# Autodesk Inventor assembly: NASA-20-FR
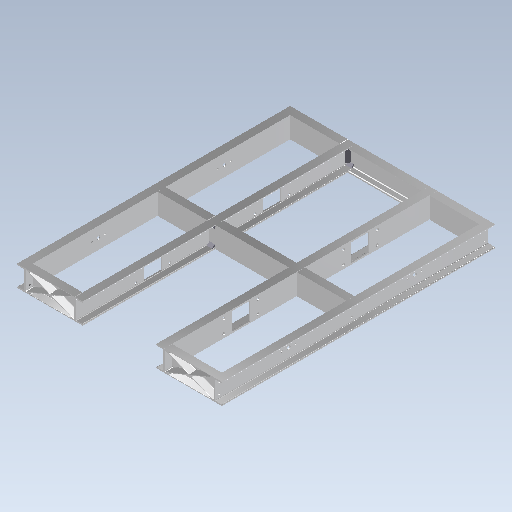
[picture p0: Inventor's stored thumbnail of the model, 512x512]
Saved by Autodesk Inventor 2020 (Build 240168000, 168)
## iProperties
Created: 2019-09-07
Part Number: NASA-20-FR
Document SubType Name: Weldment
Designer: Rick Szalay
Weld Material: Welded Aluminum-6061
Author: Rick Szalay
## Documents named in this file (6)
- C:\Users\Rick Szalay\Documents\NASA-20\NASA-20\FR\NASA-20-FR.iam
- C:\Users\Rick Szalay\Documents\NASA-20\NASA-20\FR\NASA-20-FR-SP-01.ipt
- C:\Users\Rick Szalay\Documents\NASA-20\NASA-20\FR\NASA-20-FR-BK-01.ipt
- C:\Users\Rick Szalay\Documents\NASA-20\NASA-20\FR\NASA-20-FR-FP-01.ipt
- C:\Users\Rick Szalay\Documents\NASA-20\NASA-20\FR\NASA-20-FR-TB-01.ipt
- C:\Users\Rick Szalay\Documents\NASA-20\NASA-20\FR\NASA-20-OP-01.ipt
## Components (12 placed, 5 different names)
1. NASA-20-FR-TB-01:1
2. NASA-20-FR-TB-01:2
3. NASA-20-FR-TB-01:3 — Flush:19
4. NASA-20-FR-TB-01:4
5. NASA-20-FR-TB-01:5 — Flush:18
6. NASA-20-FR-TB-01:6
7. NASA-20-FR-SP-01:1 — Mate:3, Mate:4
8. NASA-20-FR-SP-01:2 — Mate:3
9. NASA-20-FR-BK-01:1 — Flush:7, Mate:5
10. NASA-20-FR-FP-01:1 — Mate:5, Flush:18, Flush:19
11. NASA-20-OP-01:2
12. NASA-20-OP-01:1
## Relationships (35: Flush 22, Mate 13)
- [Flush]: NASA-20-FR-SP-01:1 ↔ NASA-20-FR-SP-01:2
- [Flush]: NASA-20-FR-SP-01:1 ↔ NASA-20-FR-SP-01:2
- [Flush]: NASA-20-FR-SP-01:1 ↔ NASA-20-FR-BK-01:1
- [Flush]: NASA-20-FR-SP-01:1 ↔ NASA-20-FR-BK-01:1
- [Mate]: NASA-20-FR-SP-01:1 ↔ NASA-20-FR-BK-01:1
- [Mate]: NASA-20-FR-SP-01:1 ↔ NASA-20-FR-FP-01:1
- [Flush]: NASA-20-FR-SP-01:1 ↔ NASA-20-FR-FP-01:1
- Mate:3 (-215.9 mm): NASA-20-FR-SP-01:1 ↔ NASA-20-FR-SP-01:2
- Mate:4: NASA-20-FR-SP-01:1
- Flush:7: NASA-20-FR-BK-01:1
- Mate:5 (-339.725 mm): NASA-20-FR-BK-01:1 ↔ NASA-20-FR-FP-01:1
- [Mate]: NASA-20-FR-TB-01:1 ↔ NASA-20-FR-SP-01:2
- [Flush]: NASA-20-FR-TB-01:1 ↔ NASA-20-FR-BK-01:1
- [Flush]: NASA-20-FR-TB-01:1 ↔ NASA-20-FR-SP-01:2
- [Mate]: NASA-20-FR-TB-01:3 ↔ NASA-20-FR-SP-01:2
- [Flush]: NASA-20-FR-TB-01:3 ↔ NASA-20-FR-SP-01:2
- [Mate]: NASA-20-FR-TB-01:2 ↔ NASA-20-FR-SP-01:2
- [Flush]: NASA-20-FR-TB-01:2 ↔ NASA-20-FR-SP-01:2
- [Flush]: NASA-20-FR-TB-01:2 ↔ NASA-20-FR-SP-01:2
- [Mate]: NASA-20-FR-TB-01:6 ↔ NASA-20-FR-SP-01:1
- [Mate]: NASA-20-FR-TB-01:5 ↔ NASA-20-FR-SP-01:1
- [Mate]: NASA-20-FR-TB-01:4 ↔ NASA-20-FR-SP-01:1
- [Flush]: NASA-20-FR-TB-01:5 ↔ NASA-20-FR-SP-01:1
- [Flush]: NASA-20-FR-TB-01:6 ↔ NASA-20-FR-BK-01:1
- [Flush]: NASA-20-FR-TB-01:4 ↔ NASA-20-FR-SP-01:1
- [Flush]: NASA-20-FR-TB-01:4 ↔ NASA-20-FR-SP-01:1
- [Flush]: NASA-20-FR-TB-01:6 ↔ NASA-20-FR-BK-01:1
- Flush:18: NASA-20-FR-TB-01:5 ↔ NASA-20-FR-FP-01:1
- Flush:19: NASA-20-FR-TB-01:3 ↔ NASA-20-FR-FP-01:1
- [Flush]: NASA-20-OP-01:2 ↔ NASA-20-OP-01:1
- [Flush]: NASA-20-OP-01:2 ↔ NASA-20-OP-01:1
- [Flush]: NASA-20-FR-SP-01:1 ↔ NASA-20-OP-01:1
- [Flush]: NASA-20-FR-SP-01:1 ↔ NASA-20-OP-01:1
- [Mate]: NASA-20-FR-TB-01:3 ↔ NASA-20-OP-01:2
- [Mate]: NASA-20-FR-TB-01:5 ↔ NASA-20-OP-01:1
## Named parameters: Width = 215.9 mm, Length = 660.4 mm
